# Autodesk Inventor assembly: Intake 2
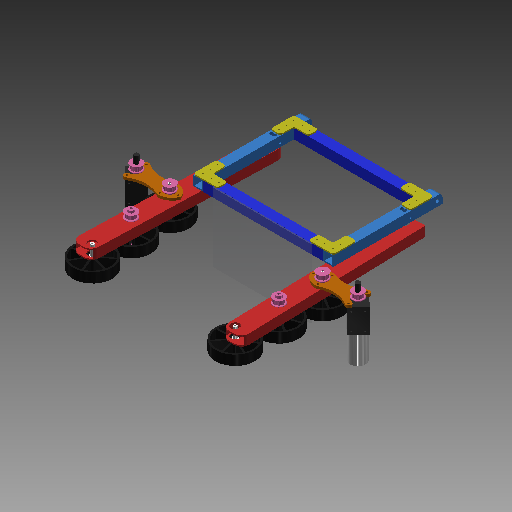
[picture p0: Inventor's stored thumbnail of the model, 512x512]
Saved by Autodesk Inventor 2017 SP1 (Build 210196100, 196)
## iProperties
Created: 2018-01-23
Part Number: Intake 2
Document SubType Name: Assembly
Designer: Ben
Mass: 3199.94 g
Surface Area: 15219.9 cm^2
Volume: 32265 cm^3
Density: 0.0991769 g/cm^3
Author: Ben
## Documents named in this file (12)
- C:\Users\Ben\Desktop\Projects\2018 Robot\Cube Intake\Intake 2.iam
- C:\Users\Ben\Desktop\Projects\2018 Robot\Cube Intake\arm.ipt
- C:\Users\Ben\Desktop\Projects\2018 Robot\Cube Intake\intake roller.ipt
- C:\Users\Ben\Desktop\Projects\2018 Robot\Cube Intake\pivot arm.ipt
- C:\Users\Ben\Desktop\Projects\2018 Robot\Cube Intake\cross brace.ipt
- C:\Users\Ben\Desktop\Projects\2018 Robot\Cube Intake\rest plate.ipt
- C:\Users\Ben\Desktop\Projects\2018 Robot\Cube Intake\micro cim.ipt
- C:\Users\Ben\Desktop\Projects\2018 Robot\Cube Intake\Part69.ipt
- C:\Users\Ben\Desktop\Projects\2018 Robot\Cube Intake\1277N450_CORROSION-RESISTANT TIMING BELT PULLEY.ipt
- C:\Users\Ben\Desktop\Projects\2018 Robot\Cube Intake\plate.ipt
- C:\Users\Ben\Desktop\Projects\2018 Robot\Cube Intake\Roller shaft.ipt
- C:\Users\Ben\Desktop\Projects\2018 Robot\Cube Intake\Roller drive shaft.ipt
## Components (37 placed, 11 different names)
1. arm:1 — Symmetry:1, Insert:1, Insert:2, Insert:3, Insert:10, Insert:15, Insert:16, Insert:27, Insert:35, Insert:36
2. arm:2 — Symmetry:1, Insert:4, Insert:5, Insert:6, Insert:7, Insert:11, Insert:12, Insert:25, Insert:37, Insert:38
3. intake roller:1 — Insert:2, Insert:30
4. intake roller:2 — Insert:1, Insert:34
5. intake roller:3 — Insert:6, Insert:23
6. intake roller:4 — Insert:4, Mate:26, Mate:27
7. intake roller:5 — Insert:5, Insert:24
8. intake roller:6 — Insert:3, Insert:29
9. pivot arm:1 — Mate:6, Mate:7, Mate:8, Flush:3, Symmetry:2, Insert:7, Mate:16, Mate:17, Flush:8, Flush:9, Mate:18, Flush:10, Mate:20, Flush:15
10. pivot arm:2 — Mate:8, Flush:3, Symmetry:2, Angle:1, Flush:4, Flush:5, Mate:10, Insert:10, Mate:19, Flush:13, Mate:21, Flush:16
11. cross brace:1 — Flush:4, Flush:5, Mate:10, Mate:11, Flush:6, Mate:16, Flush:11, Flush:12
12. rest plate:1 — Mate:11, Flush:6, Flush:7
13. micro cim:1 — Insert:14, Insert:33, Mate:24
14. Part69:1 — Insert:11, Insert:12, Insert:14, Insert:21, Insert:22, Insert:33, Mate:25
15. Part69:2 — Insert:15, Insert:16, Insert:20, Insert:31, Insert:32, Mate:23
16. micro cim:2 — Insert:31, Insert:32, Mate:22
17. 1277N450_CORROSION-RESISTANT TIMING BELT PULLEY:1 — Mate:22, Mate:23
18. 1277N450_CORROSION-RESISTANT TIMING BELT PULLEY:2 — Insert:27
19. 1277N450_CORROSION-RESISTANT TIMING BELT PULLEY:3 — Insert:34
20. 1277N450_CORROSION-RESISTANT TIMING BELT PULLEY:4 — Insert:20
21. 1277N450_CORROSION-RESISTANT TIMING BELT PULLEY:5 — Insert:21, Mate:24, Mate:25
22. 1277N450_CORROSION-RESISTANT TIMING BELT PULLEY:6 — Insert:22
23. 1277N450_CORROSION-RESISTANT TIMING BELT PULLEY:7 — Insert:25
24. 1277N450_CORROSION-RESISTANT TIMING BELT PULLEY:8 — Mate:26, Mate:27
25. 1277N450_CORROSION-RESISTANT TIMING BELT PULLEY:9 — Insert:23
26. 1277N450_CORROSION-RESISTANT TIMING BELT PULLEY:10 — Insert:24
27. 1277N450_CORROSION-RESISTANT TIMING BELT PULLEY:11 — Insert:29
28. 1277N450_CORROSION-RESISTANT TIMING BELT PULLEY:12 — Insert:30
29. cross brace:2 — Mate:17, Flush:8, Flush:9, Flush:14, Flush:17
30. plate:1 — Mate:18, Flush:10, Flush:11
31. plate:2 — Mate:19, Flush:12, Flush:13
32. plate:3 — Mate:20, Flush:14, Flush:15
33. plate:4 — Mate:21, Flush:16, Flush:17
34. Roller shaft:1 — Insert:35
35. Roller drive shaft:1 — Insert:36
36. Roller shaft:2 — Insert:37
37. Roller drive shaft:2 — Insert:38
## Relationships (65: Insert 30, Mate 17, Flush 15, Symmetry 2, Angle 1)
- Symmetry:1: arm:1 ↔ arm:2
- Insert:1 (3.175 mm): arm:1 ↔ intake roller:2
- Insert:2 (3.175 mm): arm:1 ↔ intake roller:1
- Insert:3 (3.175 mm): arm:1 ↔ intake roller:6
- Insert:4 (3.175 mm): arm:2 ↔ intake roller:4
- Insert:5 (3.175 mm): arm:2 ↔ intake roller:5
- Insert:6 (3.175 mm): arm:2 ↔ intake roller:3
- Mate:6: pivot arm:1
- Mate:7: pivot arm:1
- Mate:8: pivot arm:1 ↔ pivot arm:2
- Flush:3: pivot arm:1 ↔ pivot arm:2
- Symmetry:2: pivot arm:1 ↔ pivot arm:2
- Insert:7 (1.5875 mm): arm:2 ↔ pivot arm:1
- Angle:1 (0 deg): pivot arm:2
- Flush:4: pivot arm:2 ↔ cross brace:1
- Flush:5: pivot arm:2 ↔ cross brace:1
- Mate:10: pivot arm:2 ↔ cross brace:1
- Mate:11: cross brace:1 ↔ rest plate:1
- Flush:6: cross brace:1 ↔ rest plate:1
- Flush:7: rest plate:1
- Mate:16: pivot arm:1 ↔ cross brace:1
- Insert:10 (1.5875 mm): arm:1 ↔ pivot arm:2
- Insert:11: arm:2 ↔ Part69:1
- Insert:12: arm:2 ↔ Part69:1
- Insert:14: micro cim:1 ↔ Part69:1
- Insert:15: arm:1 ↔ Part69:2
- Insert:16: arm:1 ↔ Part69:2
- Insert:20 (1.5875 mm): Part69:2 ↔ 1277N450_CORROSION-RESISTANT TIMING BELT PULLEY:4
- Insert:21 (1.5875 mm): Part69:1 ↔ 1277N450_CORROSION-RESISTANT TIMING BELT PULLEY:5
- Insert:22 (1.5875 mm): Part69:1 ↔ 1277N450_CORROSION-RESISTANT TIMING BELT PULLEY:6
- Insert:23 (1.5875 mm): intake roller:3 ↔ 1277N450_CORROSION-RESISTANT TIMING BELT PULLEY:9
- Insert:24 (1.5875 mm): intake roller:5 ↔ 1277N450_CORROSION-RESISTANT TIMING BELT PULLEY:10
- Insert:25 (1.5875 mm): arm:2 ↔ 1277N450_CORROSION-RESISTANT TIMING BELT PULLEY:7
- Insert:27 (1.5875 mm): arm:1 ↔ 1277N450_CORROSION-RESISTANT TIMING BELT PULLEY:2
- Insert:29 (1.5875 mm): intake roller:6 ↔ 1277N450_CORROSION-RESISTANT TIMING BELT PULLEY:11
- Insert:30 (1.5875 mm): intake roller:1 ↔ 1277N450_CORROSION-RESISTANT TIMING BELT PULLEY:12
- Mate:17: pivot arm:1 ↔ cross brace:2
- Flush:8: pivot arm:1 ↔ cross brace:2
- Flush:9 (22.225 mm): pivot arm:1 ↔ cross brace:2
- Mate:18: pivot arm:1 ↔ plate:1
- Flush:10: pivot arm:1 ↔ plate:1
- Flush:11: cross brace:1 ↔ plate:1
- Mate:19: pivot arm:2 ↔ plate:2
- Flush:12: cross brace:1 ↔ plate:2
- Flush:13: pivot arm:2 ↔ plate:2
- Mate:20: pivot arm:1 ↔ plate:3
- Flush:14: cross brace:2 ↔ plate:3
- Flush:15: pivot arm:1 ↔ plate:3
- Mate:21: pivot arm:2 ↔ plate:4
- Flush:16: pivot arm:2 ↔ plate:4
- Flush:17: cross brace:2 ↔ plate:4
- Insert:31: Part69:2 ↔ micro cim:2
- Insert:32: Part69:2 ↔ micro cim:2
- Mate:22: micro cim:2 ↔ 1277N450_CORROSION-RESISTANT TIMING BELT PULLEY:1
- Mate:23 (1.5875 mm): Part69:2 ↔ 1277N450_CORROSION-RESISTANT TIMING BELT PULLEY:1
- Insert:33: micro cim:1 ↔ Part69:1
- Mate:24: micro cim:1 ↔ 1277N450_CORROSION-RESISTANT TIMING BELT PULLEY:5
- Mate:25 (1.5875 mm): Part69:1 ↔ 1277N450_CORROSION-RESISTANT TIMING BELT PULLEY:5
- Mate:26 (1.5875 mm): intake roller:4 ↔ 1277N450_CORROSION-RESISTANT TIMING BELT PULLEY:8
- Mate:27: intake roller:4 ↔ 1277N450_CORROSION-RESISTANT TIMING BELT PULLEY:8
- Insert:34 (1.5875 mm): intake roller:2 ↔ 1277N450_CORROSION-RESISTANT TIMING BELT PULLEY:3
- Insert:35 (1.5875 mm): arm:1 ↔ Roller shaft:1
- Insert:36 (1.5875 mm): arm:1 ↔ Roller drive shaft:1
- Insert:37 (1.5875 mm): arm:2 ↔ Roller shaft:2
- Insert:38 (1.5875 mm): arm:2 ↔ Roller drive shaft:2
